# Autodesk Inventor assembly: blankPC104plus
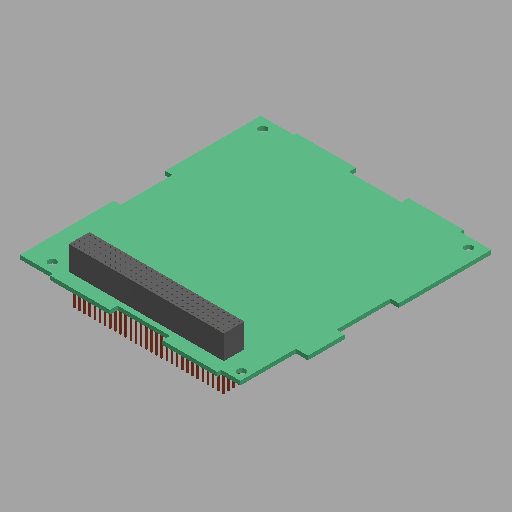
[picture p0: Inventor's stored thumbnail of the model, 512x512]
Saved by Autodesk Inventor 2022 (Build 260153000, 153)
## iProperties
Created: 2021-10-06
Part Number: blankPC104plus
Document SubType Name: Assembly
Designer: Bowen O'Steen
Author: Bowen O'Steen
## Documents named in this file (3)
- C:\Users\gwhen\OneDrive\Desktop\Vault\Designs\MEMESat\MemeSat\Engineering Data\MemeSat\Subsystems\blankPC104plus.iam
- C:\Users\gwhen\OneDrive\Desktop\Vault\Designs\MEMESat\MemeSat\Engineering Data\MemeSat\Subsystems\PC104plus.ipt
- C:\Users\gwhen\OneDrive\Desktop\Vault\Designs\MEMESat\MemeSat\Engineering Data\MemeSat\Subsystems\fullPCIconnector.iam
## Components (2 placed, 2 different names)
1. PC104plus:1 — Mate:1, Mate:2, Flush:1, Mate:3, Mate:4, Mate:5
2. fullPCIconnector:1 [sub-assembly] — Mate:3, Mate:4, Mate:5
## Relationships (6: Mate 5, Flush 1)
- Mate:1: PC104plus:1
- Mate:2: PC104plus:1
- Flush:1: PC104plus:1
- Mate:3: PC104plus:1 ↔ fullPCIconnector:1
- Mate:4: PC104plus:1 ↔ fullPCIconnector:1
- Mate:5: PC104plus:1 ↔ fullPCIconnector:1
